# Autodesk Inventor assembly: RightWheelAssembly
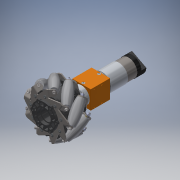
[picture p0: Inventor's stored thumbnail of the model, 180x180]
Saved by Autodesk Inventor 2018 (Build 220112000, 112)
## iProperties
Created: 2018-08-26
Part Number: RightWheelAssembly
Document SubType Name: Assembly
Designer: anirudh
Author: anirudh
## Documents named in this file (4)
- C:\Users\anirudh\Documents\MARS Fund\Silicon Edge\2018-2019\RightWheelAssembly.iam
- C:\Users\anirudh\Documents\MARS Fund\Silicon Edge\2017-2018\am-3026R4HDMecanumRightV3WithScrewsREV2.iam
- C:\Users\anirudh\Documents\MARS Fund\Silicon Edge\2017-2018\am-3639+NeveRest+Sport,+16-1+with+Motor.ipt
- C:\Users\anirudh\Documents\MARS Fund\Silicon Edge\2017-2018\FTC+Conversion+plate.ipt
## Components (3 placed, 3 different names)
1. am-3026R4HDMecanumRightV3WithScrewsREV2:1 [sub-assembly] — Angle:1, Insert:1, Angle:2
2. am-3639+NeveRest+Sport,+16-1+with+Motor:1 — Angle:3, Insert:2
3. FTC+Conversion+plate:1 — Angle:1, Insert:1, Angle:2, Angle:3, Insert:2
## Relationships (5: Angle 3, Insert 2)
- Angle:1 (0 deg): am-3026R4HDMecanumRightV3WithScrewsREV2:1 ↔ FTC+Conversion+plate:1
- Insert:1: am-3026R4HDMecanumRightV3WithScrewsREV2:1 ↔ FTC+Conversion+plate:1
- Angle:2 (8.5 deg): am-3026R4HDMecanumRightV3WithScrewsREV2:1 ↔ FTC+Conversion+plate:1
- Angle:3 (-90 deg): am-3639+NeveRest+Sport,+16-1+with+Motor:1 ↔ FTC+Conversion+plate:1
- Insert:2: am-3639+NeveRest+Sport,+16-1+with+Motor:1 ↔ FTC+Conversion+plate:1
